# Autodesk Inventor assembly: Subensamble_mesa
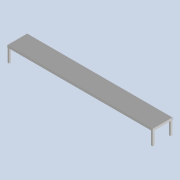
[picture p0: Inventor's stored thumbnail of the model, 180x180]
Saved by Autodesk Inventor 2021 (Build 250183000, 183)
## iProperties
Created: 2021-04-29
Part Number: Subensamble_mesa
Document SubType Name: Assembly
Designer: Admin
Author: Admin
## Documents named in this file (3)
- C:\Users\Admin\OneDrive - Universidad Nacional de Colombia\Doceabo semestre\AUTO\proyecto Auto\Proyecto_APM\CADs estaciones a automatizar\Estación corte\Subensamble_mesa.iam
- C:\Users\Admin\OneDrive - Universidad Nacional de Colombia\Doceabo semestre\AUTO\proyecto Auto\Proyecto_APM\CADs estaciones a automatizar\Estación corte\Mesa_cortadora.ipt
- C:\Users\Admin\OneDrive - Universidad Nacional de Colombia\Doceabo semestre\AUTO\proyecto Auto\Proyecto_APM\CADs estaciones a automatizar\Estación corte\Pata_mesa.ipt
## Components (5 placed, 2 different names)
1. Mesa_cortadora:1 — Coincidencia:1, Coincidencia:2, Coincidencia:3, Coincidencia:4, Coincidencia:5, Coincidencia:6, Coincidencia:7, Coincidencia:8, Coincidencia:9, Coincidencia:10, Coincidencia:11, Coincidencia:12
2. Pata_mesa:1 — Coincidencia:7, Coincidencia:8, Coincidencia:9
3. Pata_mesa:2 — Coincidencia:1, Coincidencia:2, Coincidencia:3
4. Pata_mesa:3 — Coincidencia:4, Coincidencia:5, Coincidencia:6
5. Pata_mesa:4 — Coincidencia:10, Coincidencia:11, Coincidencia:12
## Relationships (12: Mate 12)
- Coincidencia:1 [Mate]: Mesa_cortadora:1 ↔ Pata_mesa:2
- Coincidencia:2 [Mate]: Mesa_cortadora:1 ↔ Pata_mesa:2
- Coincidencia:3 [Mate]: Mesa_cortadora:1 ↔ Pata_mesa:2
- Coincidencia:4 [Mate]: Mesa_cortadora:1 ↔ Pata_mesa:3
- Coincidencia:5 [Mate]: Mesa_cortadora:1 ↔ Pata_mesa:3
- Coincidencia:6 [Mate]: Mesa_cortadora:1 ↔ Pata_mesa:3
- Coincidencia:7 [Mate]: Mesa_cortadora:1 ↔ Pata_mesa:1
- Coincidencia:8 [Mate]: Mesa_cortadora:1 ↔ Pata_mesa:1
- Coincidencia:9 [Mate]: Mesa_cortadora:1 ↔ Pata_mesa:1
- Coincidencia:10 [Mate]: Mesa_cortadora:1 ↔ Pata_mesa:4
- Coincidencia:11 [Mate]: Mesa_cortadora:1 ↔ Pata_mesa:4
- Coincidencia:12 [Mate]: Mesa_cortadora:1 ↔ Pata_mesa:4
